# Autodesk Inventor assembly: rocker_bogie_left
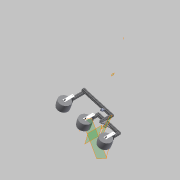
[picture p0: Inventor's stored thumbnail of the model, 180x180]
Saved by Autodesk Inventor 2021.2 (Build 252289000, 289)
## iProperties
Created: 2021-05-27
Part Number: rocker_bogie_left
Document SubType Name: Assembly
Designer: gisen
Author: gisen
## Documents named in this file (4)
- C:\Users\gisen\workspace\beetle_inventor_model\suspension\rocker_bogie_right.iam
- C:\Users\gisen\workspace\beetle_inventor_model\suspension\bogie.iam
- C:\Users\gisen\workspace\beetle_inventor_model\suspension\rocker_right.iam
- C:\Users\gisen\workspace\beetle_inventor_model\suspension\frame\ABLB-3025-6.ipt
## Components (3 placed, 3 different names)
1. bogie:1 [sub-assembly] — フラッシュ:3, 円柱状:1, フラッシュ:4, メイト:5
2. rocker_right:1 [sub-assembly] — 円柱状:1, フラッシュ:4, メイト:1, メイト:2
3. ABLB-3025-6:1 — メイト:1, メイト:2, メイト:3, 角度:1
## Relationships (9: Mate 5, Flush 2, CylindricalJoint 1, Angle 1)
- フラッシュ:3 [Flush]: bogie:1
- 円柱状:1 [CylindricalJoint]: bogie:1 ↔ rocker_right:1
- フラッシュ:4 [Flush]: bogie:1 ↔ rocker_right:1
- メイト:1 [Mate]: rocker_right:1 ↔ ABLB-3025-6:1
- メイト:2 [Mate] (-15 mm): rocker_right:1 ↔ ABLB-3025-6:1
- メイト:3 [Mate]: ABLB-3025-6:1
- メイト:4 [Mate]
- 角度:1 [Angle] (0 deg): ABLB-3025-6:1
- メイト:5 [Mate]: bogie:1
